# Autodesk Inventor assembly: wheel_MIR
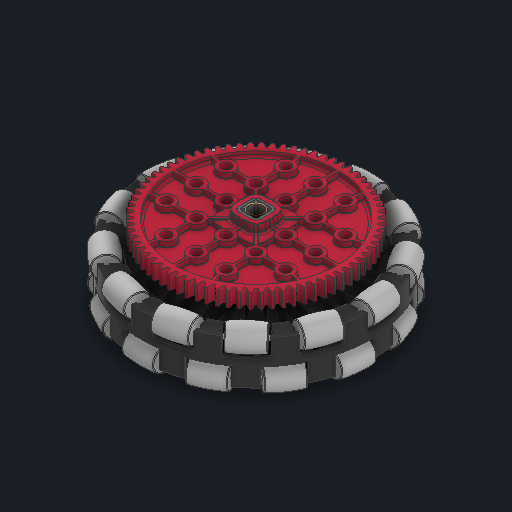
[picture p0: Inventor's stored thumbnail of the model, 512x512]
Saved by Autodesk Inventor 2024 (Build 280153000, 153)
## iProperties
Created: 2023-08-15
Part Number: wheel_MIR
Document SubType Name: Assembly
Designer: avere
Author: avere
## Documents named in this file (3)
- D:\vex_robotics\hardware\cad\scrap_v0.1\chassis\mirrored_parts\wheel_MIR.iam
- D:\vex_robotics\hardware\cad\scrap_v0.1\chassis\mirrored_parts\half_cut_72_MIR.ipt
- D:\vex_robotics\hardware\cad\scrap_v0.1\chassis\mirrored_parts\4 Omni AS, No Insert_MIR.iam
## Components (2 placed, 2 different names)
1. half_cut_72_MIR:1 — Mate:1, Insert:1
2. 4 Omni AS, No Insert_MIR:1 [sub-assembly] — Mate:1, Insert:1
## Relationships (2: Mate 1, Insert 1)
- Mate:1: half_cut_72_MIR:1 ↔ 4 Omni AS, No Insert_MIR:1
- Insert:1 (3.175 mm): half_cut_72_MIR:1 ↔ 4 Omni AS, No Insert_MIR:1
